# Autodesk Inventor assembly: Claw2017-18
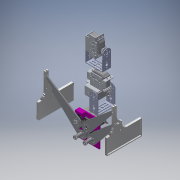
[picture p0: Inventor's stored thumbnail of the model, 180x180]
Saved by Autodesk Inventor 2017 (Build 210142000, 142)
## iProperties
Created: 2017-09-28
Part Number: Claw2017-18
Document SubType Name: Assembly
Designer: User
Author: User
## Documents named in this file (16)
- C:\Robotics\CAD\2017-18_CAD\Claw2017-18.iam
- C:\Robotics\CAD\2017-18_CAD\ClawServoHolder.ipt
- C:\Robotics\CAD\COTSParts\Tetrix\Tetrix servo 180.ipt
- C:\Robotics\CAD\COTSParts\Tetrix\Tetrix Gear 40T.ipt
- C:\Robotics\CAD\2017-18_CAD\ClawLinkage.ipt
- C:\Robotics\CAD\COTSParts\Vex\91259A576_ALLOY STEEL SHOULDER SCREW.ipt
- C:\Robotics\CAD\COTSParts\Vex\91259A581_ALLOY STEEL SHOULDER SCREW.ipt
- C:\Robotics\CAD\2017-18_CAD\ClawSpacer.ipt
- C:\Robotics\CAD\COTSParts\Tetrix\Tetrix bracket - single servo.ipt
- C:\Robotics\CAD\2017-18_CAD\TheClaw.iam
- C:\Robotics\CAD\COTSParts\Rev\REV-41-1097.ipt
- C:\Robotics\CAD\COTSParts\Tetrix\39060_txm-standard servo bracket.ipt
- C:\Robotics\CAD\COTSParts\Tetrix\39593_txm-standard-scale pivot armwbearing..ipt
- C:\Robotics\CAD\COTSParts\Tetrix\39020_txm-servo mount horn.ipt
- C:\Robotics\CAD\2017-18_CAD\2BarClawPaddle-right.ipt
- C:\Robotics\CAD\2017-18_CAD\2BarClawPaddle - left.ipt
## Components (21 placed, 15 different names)
1. ClawServoHolder:1 — Mate:5, Mate:11, Mate:12, Mate:43, Mate:44, Mate:45, Mate:46, Mate:53, Mate:54, Mate:55, Mate:58, Mate:64, Mate:78
2. Tetrix servo 180:1 — Mate:5, Mate:9, Mate:10, Mate:64, Mate:76, Mate:77, Mate:78
3. Tetrix Gear 40T:1 — Mate:9, Mate:10, Flush:5, Mate:19, Mate:20, Mate:21
4. Tetrix Gear 40T:2 — Mate:11, Mate:12, Flush:5, Mate:22, Mate:23, Mate:24
5. ClawLinkage:1 — Mate:19, Mate:20, Mate:21, Mate:87
6. ClawLinkage:2 — Mate:22, Mate:23, Mate:24, Mate:84, Mate:86
7. 91259A576_ALLOY STEEL SHOULDER SCREW:1 — Mate:43, Mate:44, Flush:6, Flush:7
8. 91259A581_ALLOY STEEL SHOULDER SCREW:3 — Mate:45, Flush:6, Mate:47, Mate:52
9. 91259A581_ALLOY STEEL SHOULDER SCREW:4 — Mate:46, Flush:7, Mate:49, Mate:51
10. ClawLinkage:3 — Mate:47, Flush:8, Mate:88, Mate:89
11. ClawLinkage:4 — Mate:49, Mate:58, Mate:85, Flush:8
12. ClawSpacer:1 — Mate:51, Mate:53
13. ClawSpacer:2 — Mate:52, Mate:54
14. Tetrix bracket - single servo:1 — Mate:55, Mate:76, Mate:77, Mate:81, Mate:82, Mate:83
15. TheClaw:1 [sub-assembly] — Mate:73, Mate:74, Mate:75
16. 39593_txm-standard-scale pivot armwbearing.:1 — Angle:1, Mate:80, Mate:81, Mate:82, Mate:83
17. 39020_txm-servo mount horn:1
18. REV-41-1097:1
19. 39060_txm-standard servo bracket:1 — Angle:1, Mate:73, Mate:74, Mate:75, Mate:80
20. 2BarClawPaddle-right:1 — Mate:84, Mate:85, Mate:86
21. 2BarClawPaddle - left:1 — Mate:87, Mate:88, Mate:89
## Relationships (50: Mate 43, Flush 4, Insert 2, Angle 1)
- Mate:5: ClawServoHolder:1 ↔ Tetrix servo 180:1
- Mate:9: Tetrix servo 180:1 ↔ Tetrix Gear 40T:1
- Mate:10: Tetrix servo 180:1 ↔ Tetrix Gear 40T:1
- Mate:11: ClawServoHolder:1 ↔ Tetrix Gear 40T:2
- Mate:12: ClawServoHolder:1 ↔ Tetrix Gear 40T:2
- Flush:5: Tetrix Gear 40T:1 ↔ Tetrix Gear 40T:2
- Mate:19: Tetrix Gear 40T:1 ↔ ClawLinkage:1
- Mate:20: Tetrix Gear 40T:1 ↔ ClawLinkage:1
- Mate:21: Tetrix Gear 40T:1 ↔ ClawLinkage:1
- Mate:22: Tetrix Gear 40T:2 ↔ ClawLinkage:2
- Mate:23: Tetrix Gear 40T:2 ↔ ClawLinkage:2
- Mate:24: Tetrix Gear 40T:2 ↔ ClawLinkage:2
- Mate:43: ClawServoHolder:1 ↔ 91259A576_ALLOY STEEL SHOULDER SCREW:1
- Mate:44: ClawServoHolder:1 ↔ 91259A576_ALLOY STEEL SHOULDER SCREW:1
- Mate:45: ClawServoHolder:1 ↔ 91259A581_ALLOY STEEL SHOULDER SCREW:3
- Flush:6: 91259A576_ALLOY STEEL SHOULDER SCREW:1 ↔ 91259A581_ALLOY STEEL SHOULDER SCREW:3
- Mate:46: ClawServoHolder:1 ↔ 91259A581_ALLOY STEEL SHOULDER SCREW:4
- Flush:7: 91259A576_ALLOY STEEL SHOULDER SCREW:1 ↔ 91259A581_ALLOY STEEL SHOULDER SCREW:4
- Mate:47: 91259A581_ALLOY STEEL SHOULDER SCREW:3 ↔ ClawLinkage:3
- Mate:49: 91259A581_ALLOY STEEL SHOULDER SCREW:4 ↔ ClawLinkage:4
- Mate:51: 91259A581_ALLOY STEEL SHOULDER SCREW:4 ↔ ClawSpacer:1
- Mate:52: 91259A581_ALLOY STEEL SHOULDER SCREW:3 ↔ ClawSpacer:2
- Mate:53: ClawServoHolder:1 ↔ ClawSpacer:1
- Mate:54: ClawServoHolder:1 ↔ ClawSpacer:2
- Mate:55 (2.54 mm): ClawServoHolder:1 ↔ Tetrix bracket - single servo:1
- Mate:58: ClawServoHolder:1 ↔ ClawLinkage:4
- Mate:64: ClawServoHolder:1 ↔ Tetrix servo 180:1
- [Mate]: 39020_txm-servo mount horn:1 ↔ REV-41-1097:1
- [Mate]: 39020_txm-servo mount horn:1 ↔ REV-41-1097:1
- [Mate]: 39593_txm-standard-scale pivot armwbearing.:1 ↔ 39060_txm-standard servo bracket:1
- [Insert]: REV-41-1097:1 ↔ 39060_txm-standard servo bracket:1
- [Insert]: REV-41-1097:1 ↔ 39060_txm-standard servo bracket:1
- Angle:1 (270 deg): 39593_txm-standard-scale pivot armwbearing.:1 ↔ 39060_txm-standard servo bracket:1
- Mate:73: TheClaw:1 ↔ 39060_txm-standard servo bracket:1
- Mate:74: TheClaw:1 ↔ 39060_txm-standard servo bracket:1
- Mate:75: TheClaw:1 ↔ 39060_txm-standard servo bracket:1
- Mate:76: Tetrix servo 180:1 ↔ Tetrix bracket - single servo:1
- Mate:77: Tetrix servo 180:1 ↔ Tetrix bracket - single servo:1
- Mate:78: ClawServoHolder:1 ↔ Tetrix servo 180:1
- Mate:80: 39593_txm-standard-scale pivot armwbearing.:1 ↔ 39060_txm-standard servo bracket:1
- Mate:81: Tetrix bracket - single servo:1 ↔ 39593_txm-standard-scale pivot armwbearing.:1
- Mate:82: Tetrix bracket - single servo:1 ↔ 39593_txm-standard-scale pivot armwbearing.:1
- Mate:83: Tetrix bracket - single servo:1 ↔ 39593_txm-standard-scale pivot armwbearing.:1
- Mate:84: ClawLinkage:2 ↔ 2BarClawPaddle-right:1
- Mate:85: ClawLinkage:4 ↔ 2BarClawPaddle-right:1
- Mate:86: ClawLinkage:2 ↔ 2BarClawPaddle-right:1
- Mate:87: ClawLinkage:1 ↔ 2BarClawPaddle - left:1
- Flush:8: ClawLinkage:3 ↔ ClawLinkage:4
- Mate:88: ClawLinkage:3 ↔ 2BarClawPaddle - left:1
- Mate:89: ClawLinkage:3 ↔ 2BarClawPaddle - left:1
## Named parameters: d130_d88 = 0 mm
